# Autodesk Inventor assembly: First_Floor
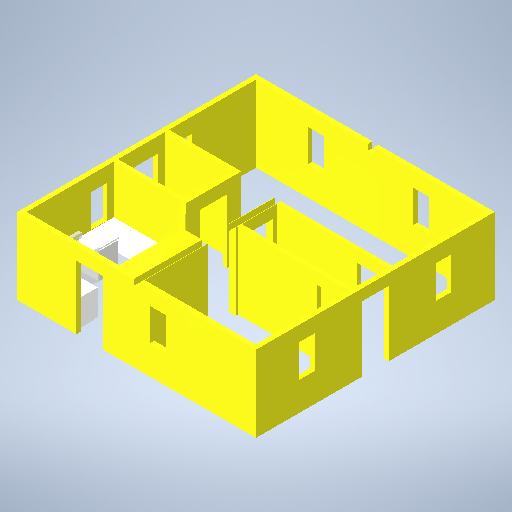
[picture p0: Inventor's stored thumbnail of the model, 512x512]
Saved by Autodesk Inventor 2025 (Build 290162000, 162)
## iProperties
Created: 2023-05-06
Part Number: First_Floor
Document SubType Name: Assembly
Designer: Tom
Author: Tom
## Documents named in this file (8)
- C:\Users\Tom\Documents\Mobility\First_Floor\Finished_First_Floor.iam
- C:\Users\Tom\Documents\Mobility\First_Floor\Walls.ipt
- C:\Users\Tom\Documents\Mobility\First_Floor\Stand_For_Sink_and_Corner_Cabinets.ipt
- C:\Users\Tom\Documents\Mobility\First_Floor\Corner_Cabinet.ipt
- C:\Users\Tom\Documents\Mobility\First_Floor\Window_Cabinet\Window_Cabinet.iam
- C:\Users\Tom\Documents\Mobility\First_Floor\Range.ipt
- C:\Users\Tom\Documents\Mobility\First_Floor\Dishwasher.ipt
- C:\Users\Tom\Documents\Mobility\First_Floor\Sink_Cabinet.ipt
## Components (7 placed, 7 different names)
1. Walls:1 — Mate:1, Mate:2, Flush:1, Mate:3, Mate:4, Mate:6, Mate:7, Flush:2, Mate:8, Flush:3, Flush:4, Mate:13
2. Stand_For_Sink_and_Corner_Cabinets:1 — Mate:1, Mate:2, Flush:1, Mate:5, Mate:14
3. Corner_Cabinet:1 — Mate:3, Mate:4, Mate:5, Mate:9, Mate:12
4. Window_Cabinet:1 [sub-assembly] — Mate:6, Mate:7, Flush:2, Mate:10, Mate:15
5. Range:1 — Mate:8, Mate:9, Flush:3
6. Dishwasher:1 — Mate:10, Flush:4, Mate:15
7. Sink_Cabinet:1 — Mate:12, Mate:13, Mate:14
## Relationships (18: Mate 14, Flush 4)
- Mate:1: Walls:1 ↔ Stand_For_Sink_and_Corner_Cabinets:1
- Mate:2: Walls:1 ↔ Stand_For_Sink_and_Corner_Cabinets:1
- Flush:1: Walls:1 ↔ Stand_For_Sink_and_Corner_Cabinets:1
- Mate:3: Walls:1 ↔ Corner_Cabinet:1
- Mate:4: Walls:1 ↔ Corner_Cabinet:1
- Mate:5: Stand_For_Sink_and_Corner_Cabinets:1 ↔ Corner_Cabinet:1
- Mate:6: Walls:1 ↔ Window_Cabinet:1
- Mate:7: Walls:1 ↔ Window_Cabinet:1
- Flush:2: Walls:1 ↔ Window_Cabinet:1
- Mate:8: Walls:1 ↔ Range:1
- Mate:9 (9.525 mm): Corner_Cabinet:1 ↔ Range:1
- Flush:3: Walls:1 ↔ Range:1
- Mate:10: Window_Cabinet:1 ↔ Dishwasher:1
- Flush:4: Walls:1 ↔ Dishwasher:1
- Mate:12: Corner_Cabinet:1 ↔ Sink_Cabinet:1
- Mate:13: Walls:1 ↔ Sink_Cabinet:1
- Mate:14: Stand_For_Sink_and_Corner_Cabinets:1 ↔ Sink_Cabinet:1
- Mate:15: Window_Cabinet:1 ↔ Dishwasher:1
